# Autodesk Inventor assembly: Ares
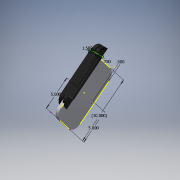
[picture p0: Inventor's stored thumbnail of the model, 180x180]
Saved by Autodesk Inventor 2018.2 (Build 222227000, 227)
## iProperties
Created: 2018-02-01
Part Number: Ares
Document SubType Name: Assembly
Designer: MIABo
Author: MIABo
## Documents named in this file (3)
- C:\Users\MIABo\OneDrive\Documents\GitHub\Ares\Ares.iam
- C:\Users\MIABo\OneDrive\Documents\GitHub\Ares\SUspension mounting.ipt
- C:\Users\MIABo\OneDrive\Documents\GitHub\Ares\Frame.ipt
## Components (2 placed, 2 different names)
1. SUspension mounting:1 — Mate:1, Mate:2
2. Frame:1 — Mate:1, Mate:2
## Relationships (2: Mate 2)
- Mate:1: SUspension mounting:1 ↔ Frame:1
- Mate:2: SUspension mounting:1 ↔ Frame:1
